# Autodesk Inventor assembly: ASY Beshkino main
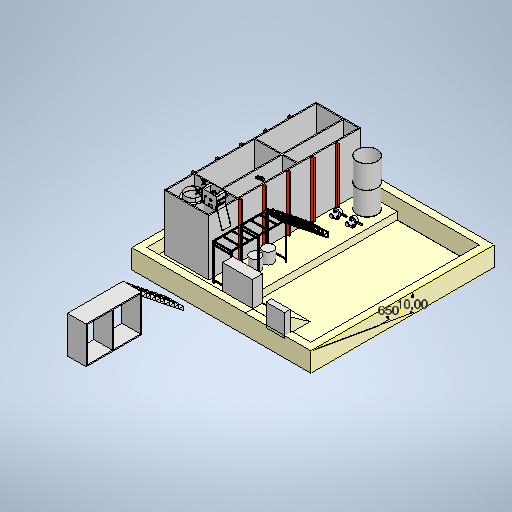
[picture p0: Inventor's stored thumbnail of the model, 512x512]
Saved by Autodesk Inventor 2025 (Build 290162010, 162A)
## iProperties
Created: 2024-08-27
Part Number: ASY Beshkino main
Document SubType Name: Assembly
Designer: DELL
Author: DELL
## Documents named in this file (17)
- C:\Users\pokla\Documents\Inventor\BSH_Beshkino_bio_tank\ASY Beshkino main.iam
- C:\Users\pokla\Documents\Inventor\BSH_Beshkino_bio_tank\BSH 0 foudation.ipt
- C:\Users\pokla\Documents\Inventor\BSH_Beshkino_bio_tank\ASY Beshkino_bio_tank.iam
- C:\Users\pokla\Documents\Inventor\BSH_Beshkino_bio_tank\ASY Trommel.iam
- C:\Users\pokla\Documents\Inventor\BSH_Beshkino_bio_tank\3d party\RXm3 assieme dimensionale mag2018.ipt
- C:\Users\pokla\Documents\Inventor\BSH_Beshkino_bio_tank\3d party\motor-reductor NMRV040\motor-reductor NMRV040.iam
- C:\Users\pokla\Documents\Inventor\BSH_Beshkino_bio_tank\BSH 01 foam filter.ipt
- C:\Users\pokla\Documents\Inventor\BSH_Beshkino_bio_tank\BSH 01 bag.ipt
- C:\Users\pokla\Documents\Inventor\BSH_Beshkino_bio_tank\BSH 03 upstairs.ipt
- C:\Users\pokla\Documents\Inventor\BSH_Beshkino_bio_tank\лестница\Перегородка\ASY NDM 11.0 перегородка.iam
- C:\Users\pokla\Documents\Inventor\BSH_Beshkino_bio_tank\Конструкция.iam
- C:\Users\pokla\Documents\Inventor\BSH_Beshkino_bio_tank\ASY BSH 500 cap.iam
- C:\Users\pokla\Documents\Inventor\BSH_Beshkino_bio_tank\ASY 080 barrel.iam
- C:\Users\pokla\Documents\Inventor\BSH_Beshkino_bio_tank\BSH 600 Tank dummy.ipt
- C:\Users\pokla\Documents\Inventor\BSH_Beshkino_bio_tank\3d party\airpump\EVL 64-41.ipt
- C:\Users\pokla\Documents\Inventor\BSH_Beshkino_bio_tank\BSH 12 reagent tank.ipt
- C:\Users\pokla\Documents\Inventor\BSH_Beshkino_bio_tank\BSH 14 elactric.ipt
## Components (19 placed, 16 different names)
1. BSH 0 foudation:1 — Mate:1, Mate:2, Mate:3, Mate:4, Flush:2, Flush:3, Flush:4, Flush:5, Mate:10, Mate:12, Mate:13, Mate:14, Mate:15, Mate:16, Mate:17, Mate:18, Flush:7
2. ASY Beshkino_bio_tank:1 [sub-assembly] — Mate:2, Mate:3, Mate:4, Mate:5, Mate:6
3. ASY Trommel:1 [sub-assembly] — Mate:9, Flush:6
4. RXm3 assieme dimensionale mag2018:1 — Mate:5
5. RXm3 assieme dimensionale mag2018:2 — Mate:6
6. motor-reductor NMRV040:1 [sub-assembly]
7. BSH 01 foam filter:1 — Flush:2, Rigid:1
8. BSH 01 bag:1 — Flush:3, Mate:14
9. BSH 03 upstairs:1 — Flush:4
10. ASY NDM 11.0 перегородка:1 [sub-assembly]
11. Конструкция:1 [sub-assembly] — Mate:10, Mate:11
12. ASY BSH 500 cap:1 [sub-assembly] — Rigid:1
13. ASY 080 barrel:1 [sub-assembly] — Mate:8
14. BSH 600 Tank dummy:1 — Flush:5, Mate:8, Mate:9, Mate:11, Mate:12, Mate:13, Flush:6
15. EVL 64-41:1 — Mate:15
16. BSH 12 reagent tank:1 — Mate:17
17. BSH 12 reagent tank:2 — Mate:16
18. EVL 64-41:2 — Mate:18
19. BSH 14 elactric:1 — Flush:7
## Relationships (24: Mate 17, Flush 6, WeldJoint 1)
- Mate:1: BSH 0 foudation:1
- Mate:2: BSH 0 foudation:1 ↔ ASY Beshkino_bio_tank:1
- Mate:3 (100 mm): BSH 0 foudation:1 ↔ ASY Beshkino_bio_tank:1
- Mate:4 (200 mm): BSH 0 foudation:1 ↔ ASY Beshkino_bio_tank:1
- Mate:5: ASY Beshkino_bio_tank:1 ↔ RXm3 assieme dimensionale mag2018:1
- Mate:6: ASY Beshkino_bio_tank:1 ↔ RXm3 assieme dimensionale mag2018:2
- Flush:2: BSH 0 foudation:1 ↔ BSH 01 foam filter:1
- Flush:3: BSH 0 foudation:1 ↔ BSH 01 bag:1
- Flush:4: BSH 0 foudation:1 ↔ BSH 03 upstairs:1
- Flush:5: BSH 0 foudation:1 ↔ BSH 600 Tank dummy:1
- Mate:8: ASY 080 barrel:1 ↔ BSH 600 Tank dummy:1
- Mate:9: ASY Trommel:1 ↔ BSH 600 Tank dummy:1
- Mate:10: BSH 0 foudation:1 ↔ Конструкция:1
- Mate:11 (120 mm): Конструкция:1 ↔ BSH 600 Tank dummy:1
- Mate:12: BSH 0 foudation:1 ↔ BSH 600 Tank dummy:1
- Mate:13 (100 mm): BSH 0 foudation:1 ↔ BSH 600 Tank dummy:1
- Flush:6: ASY Trommel:1 ↔ BSH 600 Tank dummy:1
- Mate:14: BSH 0 foudation:1 ↔ BSH 01 bag:1
- Mate:15: BSH 0 foudation:1 ↔ EVL 64-41:1
- Mate:16: BSH 0 foudation:1 ↔ BSH 12 reagent tank:2
- Mate:17: BSH 0 foudation:1 ↔ BSH 12 reagent tank:1
- Mate:18: BSH 0 foudation:1 ↔ EVL 64-41:2
- Flush:7: BSH 0 foudation:1 ↔ BSH 14 elactric:1
- Rigid:1 [WeldJoint]: BSH 01 foam filter:1 ↔ ASY BSH 500 cap:1
